# Autodesk Inventor assembly: BENCH VICE.
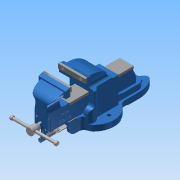
[picture p0: Inventor's stored thumbnail of the model, 180x180]
Saved by Autodesk Inventor 2014 SP1 (Build 180222100, 222)
## iProperties
Created: 2014-12-18
Part Number: BENCH VICE.
Document SubType Name: Assembly
Designer: Ebrahim
Author: Ebrahim
## Documents named in this file (14)
- D:\MY D OLD DRIVE\Ibrahim folder on Drlab216\2014-2015\BENCH VICE PACKED\Workspace\BENCH VICE..iam
- D:\MY D OLD DRIVE\Ibrahim folder on Drlab216\2014-2015\BENCH VICE PACKED\Workspace\FIXED JAW.ipt
- D:\MY D OLD DRIVE\Ibrahim folder on Drlab216\2014-2015\BENCH VICE PACKED\Workspace\MOVING JAW.ipt
- D:\MY D OLD DRIVE\Ibrahim folder on Drlab216\2014-2015\BENCH VICE PACKED\Workspace\SCREW SHAFT.ipt
- D:\MY D OLD DRIVE\Ibrahim folder on Drlab216\2014-2015\BENCH VICE PACKED\Workspace\SCREW GUIDE.ipt
- D:\MY D OLD DRIVE\Ibrahim folder on Drlab216\2014-2015\BENCH VICE PACKED\Workspace\LIVER SUBASSEMBLY.iam
- D:\MY D OLD DRIVE\Ibrahim folder on Drlab216\2014-2015\BENCH VICE PACKED\Workspace\SUPPORT PLATE.ipt
- D:\MY D OLD DRIVE\Ibrahim folder on Drlab216\2014-2015\BENCH VICE PACKED\Libraries\Content Center Files\en-US\ISO 4014(2)\ISO 4014 - M6 x 30ISO.ipt
- D:\MY D OLD DRIVE\Ibrahim folder on Drlab216\2014-2015\BENCH VICE PACKED\Libraries\Content Center Files\en-US\ISO 2009(2)\ISO 2009 - M6 x 25ISO 19.7.ipt
- D:\MY D OLD DRIVE\Ibrahim folder on Drlab216\2014-2015\BENCH VICE PACKED\Workspace\JAW CAP.ipt
- D:\MY D OLD DRIVE\Ibrahim folder on Drlab216\2014-2015\BENCH VICE PACKED\Libraries\Content Center Files\en-US\ISO 2009(2)\ISO 2009 - M8 x 20ISO 12.85.ipt
- D:\MY D OLD DRIVE\Ibrahim folder on Drlab216\2014-2015\BENCH VICE PACKED\Workspace\HANDLE.ipt
- D:\MY D OLD DRIVE\Ibrahim folder on Drlab216\2014-2015\BENCH VICE PACKED\Workspace\HANDLE CAP.ipt
- D:\MY D OLD DRIVE\Ibrahim folder on Drlab216\2014-2015\BENCH VICE PACKED\Libraries\Content Center Files\en-US\ISO 7090\ISO 7090 - 18 - 140 HV(1).ipt
## Components (19 placed, 13 different names)
1. FIXED JAW:1 — Mate:1, Flush:3, Mate:19, Mate:20, Mate:28, Mate:29, Flush:6
2. MOVING JAW:1 — Mate:1, Mate:2, Mate:12, Mate:15, Mate:18, Insert:1, Mate:24, Flush:5, Mate:25, Mate:36
3. SCREW SHAFT:1 — Mate:10, Flush:2, Insert:1, Mate:32, Flush:7
4. SCREW GUIDE:1 — Mate:11, Flush:2, Flush:3, Flush:4, Angle:1
5. LIVER SUBASSEMBLY:1 [sub-assembly] — Mate:13, Mate:14, Mate:18, Flush:4, Mate:22, Mate:23
6. SUPPORT PLATE:1 — Mate:19, Angle:1, Mate:21
7. ISO 4014 M6 x 30:1 — Mate:20, Mate:21
8. ISO 4014 M6 x 30:2
9. ISO 2009 M6 x 25 x 19.7:1 — Mate:22
10. ISO 2009 M6 x 25 x 19.7:2 — Mate:23
11. JAW CAP:1 — Mate:24, Flush:5, Mate:25, Mate:26, Mate:27
12. ISO 2009 M8 x 20 x 12.85:1 — Mate:26
13. ISO 2009 M8 x 20 x 12.85:2 — Mate:27
14. JAW CAP:2 — Mate:28, Mate:29, Flush:6, Mate:30, Mate:31
15. ISO 2009 M8 x 20 x 12.85:3 — Mate:30
16. ISO 2009 M8 x 20 x 12.85:4 — Mate:31
17. HANDLE:1 — Insert:2, Mate:33, Flush:7
18. HANDLE CAP:1 — Insert:2
19. ISO 7090 18 - 140 HV:1 — Mate:36
## Relationships (40: Mate 31, Flush 6, Insert 2, Angle 1)
- Mate:1: FIXED JAW:1 ↔ MOVING JAW:1
- Mate:2: MOVING JAW:1
- Mate:4
- Mate:6
- Mate:10: SCREW SHAFT:1
- Mate:11: SCREW GUIDE:1
- Flush:2 (312.65 mm): SCREW SHAFT:1 ↔ SCREW GUIDE:1
- Mate:12: MOVING JAW:1
- Mate:13: LIVER SUBASSEMBLY:1
- Mate:14: LIVER SUBASSEMBLY:1
- Mate:15: MOVING JAW:1
- Mate:16
- Mate:17
- Mate:18: MOVING JAW:1 ↔ LIVER SUBASSEMBLY:1
- Insert:1: MOVING JAW:1 ↔ SCREW SHAFT:1
- Flush:3 (-1 mm): FIXED JAW:1 ↔ SCREW GUIDE:1
- Flush:4 (2 mm): SCREW GUIDE:1 ↔ LIVER SUBASSEMBLY:1
- Mate:19: FIXED JAW:1 ↔ SUPPORT PLATE:1
- Angle:1 (90 deg): SCREW GUIDE:1 ↔ SUPPORT PLATE:1
- Mate:20: FIXED JAW:1 ↔ ISO 4014 M6 x 30:1
- Mate:21: SUPPORT PLATE:1 ↔ ISO 4014 M6 x 30:1
- Mate:22: LIVER SUBASSEMBLY:1 ↔ ISO 2009 M6 x 25 x 19.7:1
- Mate:23: LIVER SUBASSEMBLY:1 ↔ ISO 2009 M6 x 25 x 19.7:2
- Mate:24: MOVING JAW:1 ↔ JAW CAP:1
- Flush:5 (-0.461 mm): MOVING JAW:1 ↔ JAW CAP:1
- Mate:25: MOVING JAW:1 ↔ JAW CAP:1
- Mate:26: JAW CAP:1 ↔ ISO 2009 M8 x 20 x 12.85:1
- Mate:27: JAW CAP:1 ↔ ISO 2009 M8 x 20 x 12.85:2
- Mate:28: FIXED JAW:1 ↔ JAW CAP:2
- Mate:29: FIXED JAW:1 ↔ JAW CAP:2
- Flush:6: FIXED JAW:1 ↔ JAW CAP:2
- Mate:30: JAW CAP:2 ↔ ISO 2009 M8 x 20 x 12.85:3
- Mate:31: JAW CAP:2 ↔ ISO 2009 M8 x 20 x 12.85:4
- Insert:2 (-14 mm): HANDLE:1 ↔ HANDLE CAP:1
- Mate:32: SCREW SHAFT:1
- Mate:33: HANDLE:1
- Mate:34
- Flush:7: SCREW SHAFT:1 ↔ HANDLE:1
- [Mate]: SCREW SHAFT:1 ↔ ISO 7090 18 - 140 HV:1
- Mate:36: MOVING JAW:1 ↔ ISO 7090 18 - 140 HV:1
